# Autodesk Inventor assembly: IOT-Trike
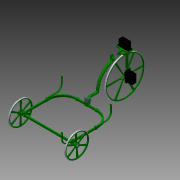
[picture p0: Inventor's stored thumbnail of the model, 180x180]
Saved by Autodesk Inventor 2014 SP1 (Build 180222100, 222)
## iProperties
Created: 2017-01-18
Part Number: IOT-Trike
Document SubType Name: Assembly
Designer: danielsikar
Author: danielsikar
## Documents named in this file (6)
- C:\Users\danielsikar\Documents\Inventor\IoT-Trike\Assemblies\IOT-Trike.iam
- C:\Users\danielsikar\Documents\Inventor\IoT-Trike\Assemblies\BackAxlePlusWheels.iam
- C:\Users\danielsikar\Documents\Inventor\IoT-Trike\Assemblies\ForkHandleBar.iam
- C:\Users\danielsikar\Documents\Inventor\IoT-Trike\Assemblies\Undercarriage.iam
- C:\Users\danielsikar\Documents\Inventor\IoT-Trike\Parts\MudGuard.ipt
- C:\Users\danielsikar\Documents\Inventor\IoT-Trike\Parts\MudGuardBrace.ipt
## Components (5 placed, 5 different names)
1. BackAxlePlusWheels:1 [sub-assembly] — Flush:1, Mate:1, Mate:2, Mate:4, Mate:5, Mate:6
2. ForkHandleBar:1 [sub-assembly] — Flush:2, Mate:3
3. Undercarriage:1 [sub-assembly] — Mate:4, Mate:5, Mate:6, Mate:7, Flush:3, Mate:8, Mate:9
4. MudGuard:1 — Mate:7, Flush:3, Mate:8, Flush:4, Flush:5
5. MudGuardBrace:1 — Flush:4, Flush:5, Mate:9
## Relationships (14: Mate 9, Flush 5)
- Flush:1: BackAxlePlusWheels:1
- Mate:1: BackAxlePlusWheels:1
- Mate:2: BackAxlePlusWheels:1
- Flush:2: ForkHandleBar:1
- Mate:3 (139.25 mm): ForkHandleBar:1
- Mate:4: BackAxlePlusWheels:1 ↔ Undercarriage:1
- Mate:5: BackAxlePlusWheels:1 ↔ Undercarriage:1
- Mate:6: BackAxlePlusWheels:1 ↔ Undercarriage:1
- Mate:7: Undercarriage:1 ↔ MudGuard:1
- Flush:3: Undercarriage:1 ↔ MudGuard:1
- Mate:8: Undercarriage:1 ↔ MudGuard:1
- Flush:4: MudGuard:1 ↔ MudGuardBrace:1
- Flush:5: MudGuard:1 ↔ MudGuardBrace:1
- Mate:9: Undercarriage:1 ↔ MudGuardBrace:1
